# Autodesk Inventor assembly: 2024-000
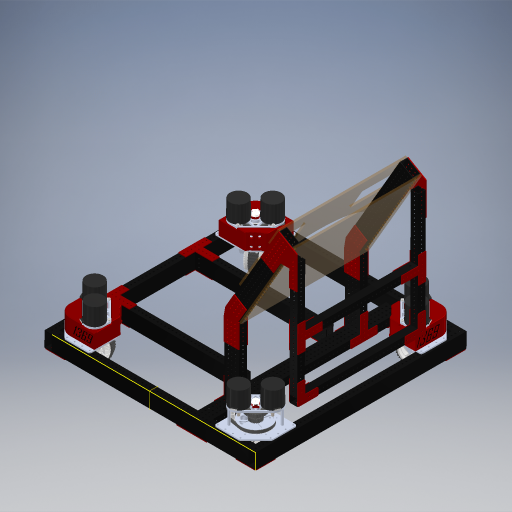
[picture p0: Inventor's stored thumbnail of the model, 512x512]
Saved by Autodesk Inventor 2024.2 (Build 282272000, 272)
## iProperties
Created: 2024-01-07
Part Number: 2024-000
Document SubType Name: Assembly
Designer: rohan
Author: rohan
## Documents named in this file (4)
- C:\Users\rohan\OneDrive - Hillsborough County Public Schools\Robotics\FIRST-Robotics-Competition\Crescendo\Minotaur-Crescendo-Robot\2024-000.iam
- C:\Users\rohan\OneDrive - Hillsborough County Public Schools\Robotics\FIRST-Robotics-Competition\Crescendo\Minotaur-Crescendo-Robot\Swerve-Drivetrain.iam
- C:\Users\rohan\OneDrive - Hillsborough County Public Schools\Robotics\FIRST-Robotics-Competition\Crescendo\Minotaur-Crescendo-Robot\Structure\Superstructure\Fixed Shooter\2024-210-Fixed-Shootaur.iam
- C:\Users\rohan\OneDrive - Hillsborough County Public Schools\Robotics\FIRST-Robotics-Competition\Crescendo\Minotaur-Crescendo-Robot\Structure\Gussets\THRIFYBOT-T-Gusset.ipt
## Components (6 placed, 3 different names)
1. Swerve-Drivetrain:1 [sub-assembly] — Tangent:1, Flush:1, Flush:4, Mate:4, Insert:1, Flush:8, Insert:3
2. 2024-210-Fixed-Shootaur:1 [sub-assembly] — Flush:1, Mate:3, Mate:4, Insert:2, Mate:6, Flush:7, Insert:4
3. THRIFYBOT-T-Gusset:1 — Flush:2, Flush:3, Mate:2
4. THRIFYBOT-T-Gusset:2 — Flush:2, Flush:3, Mate:2, Mate:3, Flush:4, Insert:1, Insert:2
5. THRIFYBOT-T-Gusset:3
6. THRIFYBOT-T-Gusset:4 — Mate:6, Flush:7, Flush:8, Insert:3, Insert:4
## Relationships (18: Flush 8, Mate 5, Insert 4, Tangent 1)
- Tangent:1: Swerve-Drivetrain:1
- Flush:1: Swerve-Drivetrain:1 ↔ 2024-210-Fixed-Shootaur:1
- Flush:2: THRIFYBOT-T-Gusset:1 ↔ THRIFYBOT-T-Gusset:2
- Flush:3: THRIFYBOT-T-Gusset:1 ↔ THRIFYBOT-T-Gusset:2
- Mate:2 (50.8 mm): THRIFYBOT-T-Gusset:1 ↔ THRIFYBOT-T-Gusset:2
- Mate:3: 2024-210-Fixed-Shootaur:1 ↔ THRIFYBOT-T-Gusset:2
- Flush:4: Swerve-Drivetrain:1 ↔ THRIFYBOT-T-Gusset:2
- Mate:4: Swerve-Drivetrain:1 ↔ 2024-210-Fixed-Shootaur:1
- Insert:1: Swerve-Drivetrain:1 ↔ THRIFYBOT-T-Gusset:2
- Insert:2: 2024-210-Fixed-Shootaur:1 ↔ THRIFYBOT-T-Gusset:2
- [Flush]: THRIFYBOT-T-Gusset:3 ↔ THRIFYBOT-T-Gusset:4
- [Flush]: THRIFYBOT-T-Gusset:3 ↔ THRIFYBOT-T-Gusset:4
- [Mate] (50.8 mm): THRIFYBOT-T-Gusset:3 ↔ THRIFYBOT-T-Gusset:4
- Mate:6: 2024-210-Fixed-Shootaur:1 ↔ THRIFYBOT-T-Gusset:4
- Flush:7: 2024-210-Fixed-Shootaur:1 ↔ THRIFYBOT-T-Gusset:4
- Flush:8: Swerve-Drivetrain:1 ↔ THRIFYBOT-T-Gusset:4
- Insert:3: Swerve-Drivetrain:1 ↔ THRIFYBOT-T-Gusset:4
- Insert:4: 2024-210-Fixed-Shootaur:1 ↔ THRIFYBOT-T-Gusset:4
## Named parameters: d132_d120 = 0 mm, d133_d121 = 0 mm, d134_d122 = 50.8 mm
